# Autodesk Inventor assembly: Inner Channel
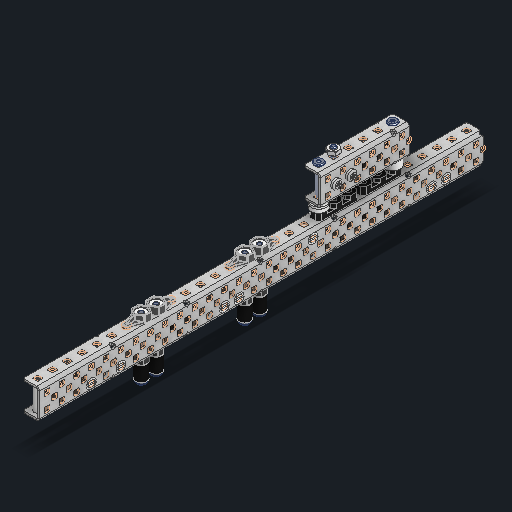
[picture p0: Inventor's stored thumbnail of the model, 512x512]
Saved by Autodesk Inventor 2025.1 (Build 291241000, 241)
## iProperties
Created: 2024-11-04
Part Number: Inner Channel
Document SubType Name: Assembly
Designer: avere
Author: avere
## Documents named in this file (27)
- C:\Users\avere\VEX\High Stakes\CAD\V3\Chassis\Drivebay Left\Inner Channel.iam
- C:\Users\avere\VEX\High Stakes\CAD\ROBOPROS-CAD-Inventor\Structure\C Channel\Aluminum 1x2x1\Alu C 1x2x1x30.ipt
- C:\Users\avere\VEX\High Stakes\CAD\ROBOPROS-CAD-Inventor\Quick Assemblies\Bearing Flat NScrew Slotted.iam
- C:\Users\avere\VEX\High Stakes\CAD\ROBOPROS-CAD-Inventor\Motion\Spacers\Spacer Nylon .375 OD.ipt
- C:\Users\avere\VEX\High Stakes\CAD\ROBOPROS-CAD-Inventor\Structure\C Channel\Aluminum 1x2x1\Alu C 1x2x1x6.ipt
- C:\Users\avere\VEX\High Stakes\CAD\ROBOPROS-CAD-Inventor\Motion\Shaft LS\Bearing Flat.ipt
- C:\Users\avere\VEX\High Stakes\CAD\ROBOPROS-CAD-Inventor\Motion\Spacers\Spacer Nylon .500 OD\NSpacer White .500 OD x .250.ipt
- C:\Users\avere\VEX\High Stakes\CAD\ROBOPROS-CAD-Inventor\Motion\Spacers\Spacer Nylon .500 OD.ipt
- C:\Users\avere\VEX\High Stakes\CAD\ROBOPROS-CAD-Inventor\Quick Assemblies\Bearing Flat NScrew Slotted Offset.iam
- C:\Users\avere\VEX\High Stakes\CAD\ROBOPROS-CAD-Inventor\Structure\Hardware\Screw Steel - Star\SScrew Star Smooth 1.750.ipt
- C:\Users\avere\VEX\High Stakes\CAD\ROBOPROS-CAD-Inventor\Structure\Hardware\Screw Steel - Star.ipt
- C:\Users\avere\VEX\High Stakes\CAD\ROBOPROS-CAD-Inventor\Structure\Hardware\Screw Steel - Star\SScrew Star Smooth .250.ipt
- C:\Users\avere\VEX\High Stakes\CAD\ROBOPROS-CAD-Inventor\Structure\Nylon Standoff Rounded\Nylon Standoff .875.ipt
- C:\Users\avere\VEX\High Stakes\CAD\ROBOPROS-CAD-Inventor\Motion\Spacers\Spacer Nylon .375 OD\NSpacer .375 OD x .500.ipt
- C:\Users\avere\VEX\High Stakes\CAD\ROBOPROS-CAD-Inventor\Structure\Hardware\Nut Nylon\Nut Nylon - White.ipt
- C:\Users\avere\VEX\High Stakes\CAD\ROBOPROS-CAD-Inventor\Structure\Hardware\Nut Nylon.ipt
- C:\Users\avere\VEX\High Stakes\CAD\ROBOPROS-CAD-Inventor\Structure\Hardware\Screw Shoulder Robosource\SScrew Shoulder Smooth 2.000 x .04.ipt
- C:\Users\avere\VEX\High Stakes\CAD\ROBOPROS-CAD-Inventor\Structure\Hardware\Screw Shoulder Robosource.ipt
- C:\Users\avere\VEX\High Stakes\CAD\ROBOPROS-CAD-Inventor\Modified Parts\Bearing Flat Low Profile 2-Hole.ipt
- C:\Users\avere\VEX\High Stakes\CAD\ROBOPROS-CAD-Inventor\Structure\1-Post Hex Nut Retainer With Nylon Hardware.iam
- C:\Users\avere\VEX\High Stakes\CAD\V3\Chassis\Drivebay Left\Nut Nylon Thread-Forming.ipt
- C:\Users\avere\VEX\High Stakes\CAD\ROBOPROS-CAD-Inventor\Structure\Hardware\Screw Nylon - Slotted\NScrew Slotted Threaded .500.ipt
- C:\Users\avere\VEX\High Stakes\CAD\ROBOPROS-CAD-Inventor\Structure\Hardware\Screw Nylon - Pan Head\NScrew Pan Head Threaded .250.ipt
- C:\Users\avere\VEX\High Stakes\CAD\ROBOPROS-CAD-Inventor\Structure\Hardware\Screw Shoulder Robosource\SScrew Shoulder Smooth .375 x .12.ipt
- C:\Users\avere\VEX\High Stakes\CAD\ROBOPROS-CAD-Inventor\Motion\Spacers\Spacer Nylon .500 OD\NSpacer White .500 OD x .125.ipt
- C:\Users\avere\VEX\High Stakes\CAD\ROBOPROS-CAD-Inventor\Motion\Spacers\Washer Steel\SWasher .500 OD x .062500\SWasher .500 OD x .062500.ipt
- C:\Users\avere\VEX\High Stakes\CAD\ROBOPROS-CAD-Inventor\Motion\Spacers\Washer Steel\SWasher .500 OD x .062500.ipt
## Components (52 placed, 20 different names)
1. Alu C 1x2x1x30:1 — Flush:1, Flush:2, Flush:3, Insert:44, Insert:45, Insert:46, Insert:47, Insert:50, Mate:15, Insert:55, Insert:56, Mate:17, Insert:58, Mate:19, Insert:59, Mate:20, Insert:61, Insert:62, Mate:21, Insert:63, Insert:67, Insert:68, Insert:69, Insert:74, Mate:25, Insert:75, Insert:76, Insert:77, Insert:78, Insert:79, Insert:80, Insert:84, Mate:28, Insert:85, Mate:29, Insert:86, Insert:88, Insert:89, Insert:94, Insert:95
2. Bearing Flat NScrew Slotted Offset:2 [sub-assembly] — Insert:59, Mate:20
3. Bearing Flat NScrew Slotted:8 [sub-assembly] — Insert:58, Mate:19
4. Nylon Standoff .875:3 — Insert:67
5. Nylon Standoff .875:4 — Insert:68
6. Nylon Standoff .875:5 — Insert:69
7. Nut Nylon Thread-Forming:1 — Insert:102
8. Nut Nylon Thread-Forming:2 — Insert:103
9. Bearing Flat NScrew Slotted Offset:3 [sub-assembly] — Insert:84, Mate:28
10. Bearing Flat Low Profile 2-Hole:3 — Insert:85, Mate:29, Insert:87
11. NScrew Slotted Threaded .500:1 — Insert:86
12. Nut Nylon - White:10 — Insert:87
13. Nut Nylon - White:11 — Insert:89
14. Nut Nylon - White:12 — Insert:88
15. NScrew Pan Head Threaded .250:1 — Insert:92
16. NScrew Pan Head Threaded .250:2 — Insert:91
17. Nylon Standoff .875:6 — Insert:94
18. SScrew Star Smooth .250:4 — Insert:95
19. SScrew Star Smooth 1.750:5 — Insert:93
20. SScrew Shoulder Smooth .375 x .12:5 — Insert:96
21. Nut Nylon Thread-Forming:3 — Insert:101
22. NSpacer White .500 OD x .125:3 — Insert:99
23. SWasher .500 OD x .062500:1 — Insert:100
24. SScrew Star Smooth 1.750:2 — Insert:61
25. SScrew Star Smooth .250:3 — Insert:32
26. Alu C 1x2x1x6:1 — Insert:32, Insert:39, Insert:64, Insert:91, Insert:92, Insert:93, Insert:96, Insert:100, Insert:101, Insert:102, Insert:103
27. Bearing Flat:1 — Insert:62, Mate:21, Insert:99
28. Bearing Flat:2 — Insert:20, Insert:63
29. NSpacer White .500 OD x .250:2 — Insert:20, Insert:64
30. Nylon Standoff .875:2 — Insert:39
31. NSpacer .375 OD x .500:5 — Insert:51, Insert:54
32. NSpacer .375 OD x .500:7 — Insert:52, Insert:53
33. Nut Nylon - White:1 — Insert:45
34. Nut Nylon - White:2 — Insert:44
35. Nut Nylon - White:3 — Insert:46
36. Nut Nylon - White:4 — Insert:47
37. SScrew Shoulder Smooth 2.000 x .04:1 — Insert:53, Mate:16
38. SScrew Shoulder Smooth 2.000 x .04:2 — Insert:54
39. Bearing Flat Low Profile 2-Hole:1 — Insert:50, Mate:15, Insert:51, Insert:52
40. 1-Post Hex Nut Retainer With Nylon Hardware:1 [sub-assembly] — Insert:55, Mate:16
41. 1-Post Hex Nut Retainer With Nylon Hardware:2 [sub-assembly] — Insert:56, Mate:17
42. NSpacer .375 OD x .500:8
43. NSpacer .375 OD x .500:9
44. Nut Nylon - White:5 — Insert:76
45. Nut Nylon - White:6 — Insert:77
46. Nut Nylon - White:7 — Insert:75
47. SScrew Shoulder Smooth 2.000 x .04:3
48. SScrew Shoulder Smooth 2.000 x .04:4 — Mate:26
49. Bearing Flat Low Profile 2-Hole:2 — Insert:74, Mate:25
50. 1-Post Hex Nut Retainer With Nylon Hardware:3 [sub-assembly] — Insert:79
51. 1-Post Hex Nut Retainer With Nylon Hardware:4 [sub-assembly] — Insert:80, Mate:26
52. Nut Nylon - White:9 — Insert:78
## Relationships (66: Insert 52, Mate 11, Flush 3)
- Flush:1 (-190.5 mm): Alu C 1x2x1x30:1
- Flush:2 (-38.1 mm): Alu C 1x2x1x30:1
- Flush:3 (-7.9375 mm): Alu C 1x2x1x30:1
- Insert:20: Bearing Flat:2 ↔ NSpacer White .500 OD x .250:2
- Insert:32: SScrew Star Smooth .250:3 ↔ Alu C 1x2x1x6:1
- Insert:39: Alu C 1x2x1x6:1 ↔ Nylon Standoff .875:2
- Insert:44: Alu C 1x2x1x30:1 ↔ Nut Nylon - White:2
- Insert:45: Alu C 1x2x1x30:1 ↔ Nut Nylon - White:1
- Insert:46: Alu C 1x2x1x30:1 ↔ Nut Nylon - White:3
- Insert:47: Alu C 1x2x1x30:1 ↔ Nut Nylon - White:4
- Insert:50: Alu C 1x2x1x30:1 ↔ Bearing Flat Low Profile 2-Hole:1
- Mate:15: Alu C 1x2x1x30:1 ↔ Bearing Flat Low Profile 2-Hole:1
- Insert:51 (1.27 mm): NSpacer .375 OD x .500:5 ↔ Bearing Flat Low Profile 2-Hole:1
- Insert:52 (1.27 mm): NSpacer .375 OD x .500:7 ↔ Bearing Flat Low Profile 2-Hole:1
- Insert:53 (1.5875 mm): NSpacer .375 OD x .500:7 ↔ SScrew Shoulder Smooth 2.000 x .04:1
- Insert:54 (1.5875 mm): NSpacer .375 OD x .500:5 ↔ SScrew Shoulder Smooth 2.000 x .04:2
- Insert:55: Alu C 1x2x1x30:1 ↔ 1-Post Hex Nut Retainer With Nylon Hardware:1
- Mate:16: SScrew Shoulder Smooth 2.000 x .04:1 ↔ 1-Post Hex Nut Retainer With Nylon Hardware:1
- Insert:56: Alu C 1x2x1x30:1 ↔ 1-Post Hex Nut Retainer With Nylon Hardware:2
- Mate:17: Alu C 1x2x1x30:1 ↔ 1-Post Hex Nut Retainer With Nylon Hardware:2
- Insert:58: Alu C 1x2x1x30:1 ↔ Bearing Flat NScrew Slotted:8
- Mate:19: Alu C 1x2x1x30:1 ↔ Bearing Flat NScrew Slotted:8
- Insert:59: Alu C 1x2x1x30:1 ↔ Bearing Flat NScrew Slotted Offset:2
- Mate:20: Alu C 1x2x1x30:1 ↔ Bearing Flat NScrew Slotted Offset:2
- Insert:61: Alu C 1x2x1x30:1 ↔ SScrew Star Smooth 1.750:2
- Insert:62: Alu C 1x2x1x30:1 ↔ Bearing Flat:1
- Mate:21: Alu C 1x2x1x30:1 ↔ Bearing Flat:1
- Insert:63: Alu C 1x2x1x30:1 ↔ Bearing Flat:2
- Insert:64: Alu C 1x2x1x6:1 ↔ NSpacer White .500 OD x .250:2
- Insert:67: Alu C 1x2x1x30:1 ↔ Nylon Standoff .875:3
- Insert:68: Alu C 1x2x1x30:1 ↔ Nylon Standoff .875:4
- Insert:69: Alu C 1x2x1x30:1 ↔ Nylon Standoff .875:5
- [Insert] (1.27 mm): NSpacer .375 OD x .500:8 ↔ Bearing Flat Low Profile 2-Hole:2
- [Insert] (1.27 mm): NSpacer .375 OD x .500:9 ↔ Bearing Flat Low Profile 2-Hole:2
- [Insert] (1.5875 mm): NSpacer .375 OD x .500:9 ↔ SScrew Shoulder Smooth 2.000 x .04:3
- [Insert] (1.5875 mm): NSpacer .375 OD x .500:8 ↔ SScrew Shoulder Smooth 2.000 x .04:4
- [Mate]: SScrew Shoulder Smooth 2.000 x .04:3 ↔ 1-Post Hex Nut Retainer With Nylon Hardware:3
- Insert:74: Alu C 1x2x1x30:1 ↔ Bearing Flat Low Profile 2-Hole:2
- Mate:25: Alu C 1x2x1x30:1 ↔ Bearing Flat Low Profile 2-Hole:2
- Insert:75: Alu C 1x2x1x30:1 ↔ Nut Nylon - White:7
- Insert:76: Alu C 1x2x1x30:1 ↔ Nut Nylon - White:5
- Insert:77: Alu C 1x2x1x30:1 ↔ Nut Nylon - White:6
- Insert:78: Alu C 1x2x1x30:1 ↔ Nut Nylon - White:9
- Insert:79: Alu C 1x2x1x30:1 ↔ 1-Post Hex Nut Retainer With Nylon Hardware:3
- Insert:80: Alu C 1x2x1x30:1 ↔ 1-Post Hex Nut Retainer With Nylon Hardware:4
- Mate:26: SScrew Shoulder Smooth 2.000 x .04:4 ↔ 1-Post Hex Nut Retainer With Nylon Hardware:4
- Insert:84: Alu C 1x2x1x30:1 ↔ Bearing Flat NScrew Slotted Offset:3
- Mate:28: Alu C 1x2x1x30:1 ↔ Bearing Flat NScrew Slotted Offset:3
- Insert:85: Alu C 1x2x1x30:1 ↔ Bearing Flat Low Profile 2-Hole:3
- Mate:29: Alu C 1x2x1x30:1 ↔ Bearing Flat Low Profile 2-Hole:3
- Insert:86: Alu C 1x2x1x30:1 ↔ NScrew Slotted Threaded .500:1
- Insert:87 (1.27 mm): Bearing Flat Low Profile 2-Hole:3 ↔ Nut Nylon - White:10
- Insert:88: Alu C 1x2x1x30:1 ↔ Nut Nylon - White:12
- Insert:89: Alu C 1x2x1x30:1 ↔ Nut Nylon - White:11
- Insert:91: NScrew Pan Head Threaded .250:2 ↔ Alu C 1x2x1x6:1
- Insert:92: NScrew Pan Head Threaded .250:1 ↔ Alu C 1x2x1x6:1
- Insert:93 (1.5875 mm): SScrew Star Smooth 1.750:5 ↔ Alu C 1x2x1x6:1
- Insert:94: Alu C 1x2x1x30:1 ↔ Nylon Standoff .875:6
- Insert:95: Alu C 1x2x1x30:1 ↔ SScrew Star Smooth .250:4
- Insert:96: SScrew Shoulder Smooth .375 x .12:5 ↔ Alu C 1x2x1x6:1
- [Insert]: NSpacer White .500 OD x .125:3 ↔ SWasher .500 OD x .062500:1
- Insert:99: NSpacer White .500 OD x .125:3 ↔ Bearing Flat:1
- Insert:100 (1.5875 mm): SWasher .500 OD x .062500:1 ↔ Alu C 1x2x1x6:1
- Insert:101 (3.175 mm): Nut Nylon Thread-Forming:3 ↔ Alu C 1x2x1x6:1
- Insert:102: Nut Nylon Thread-Forming:1 ↔ Alu C 1x2x1x6:1
- Insert:103: Nut Nylon Thread-Forming:2 ↔ Alu C 1x2x1x6:1
## Named parameters: d235_d194 = 1.27 mm, d236_d195 = 1.27 mm, d237_d196 = 1.5875 mm, d238_d197 = 1.5875 mm, d239_d199 = 0 mm, d274_d255 = 0 mm
